# Autodesk Inventor assembly: Cold Plate
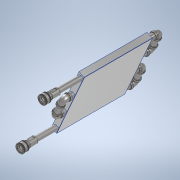
[picture p0: Inventor's stored thumbnail of the model, 180x180]
Saved by Autodesk Inventor 2022 (Build 260153000, 153)
## iProperties
Created: 2022-01-20
Part Number: Cold Plate
Document SubType Name: Assembly
Designer: Caleb
Author: Caleb
## Documents named in this file (8)
- C:\Users\Caleb\Desktop\nebraska-silicon-lab\Hardware\TFPX\Cold Plate\Cold Plate.iam
- C:\Users\Caleb\Desktop\nebraska-silicon-lab\Hardware\TFPX\Cold Plate\43685K12_Low-Pressure Socket-Connect Unthreaded Pipe Fitting.ipt
- C:\Users\Caleb\Desktop\nebraska-silicon-lab\Hardware\TFPX\Cold Plate\outer pipe section.ipt
- C:\Users\Caleb\Desktop\nebraska-silicon-lab\Hardware\TFPX\Cold Plate\inner pipe section.ipt
- C:\Users\Caleb\Desktop\nebraska-silicon-lab\Hardware\TFPX\Cold Plate\Plate.ipt
- C:\Users\Caleb\Desktop\nebraska-silicon-lab\Hardware\TFPX\Cold Plate\5341K26_Pioneer Quick-Disconnect Hose Coupling for Hydraulic Fluid.ipt
- C:\Users\Caleb\Desktop\nebraska-silicon-lab\Hardware\TFPX\Cold Plate\Cover.ipt
- C:\Users\Caleb\Desktop\nebraska-silicon-lab\Hardware\TFPX\Cold Plate\long inner pipe section threaded.ipt
## Components (17 placed, 7 different names)
1. 43685K12_Low-Pressure Socket-Connect Unthreaded Pipe Fitting:1 — Insert:1, Insert:2, Flush:1
2. outer pipe section:1 — Insert:2, Insert:3
3. outer pipe section:2 — Insert:6, Insert:7
4. inner pipe section:1 — Insert:4, Insert:5, Mate:3
5. inner pipe section:2 — Insert:1, Insert:9
6. 43685K12_Low-Pressure Socket-Connect Unthreaded Pipe Fitting:2 — Insert:3, Flush:1, Insert:4
7. 43685K12_Low-Pressure Socket-Connect Unthreaded Pipe Fitting:3 — Insert:5, Insert:6
8. 43685K12_Low-Pressure Socket-Connect Unthreaded Pipe Fitting:4 — Insert:7, Mate:2, Insert:13
9. 43685K12_Low-Pressure Socket-Connect Unthreaded Pipe Fitting:5 — Insert:9, Insert:10
10. 43685K12_Low-Pressure Socket-Connect Unthreaded Pipe Fitting:6 — Insert:11, Insert:12
11. outer pipe section:3 — Insert:10, Insert:11
12. Plate:1 — Mate:2, Mate:3, Mate:4, Flush:2, Flush:3
13. 5341K26_Pioneer Quick-Disconnect Hose Coupling for Hydraulic Fluid:1 — Insert:14
14. 5341K26_Pioneer Quick-Disconnect Hose Coupling for Hydraulic Fluid:2 — Insert:15
15. long inner pipe section threaded:1 — Insert:12, Insert:14
16. long inner pipe section threaded:2 — Insert:13, Insert:15
17. Cover:1 — Mate:4, Flush:2, Flush:3
## Relationships (20: Insert 14, Flush 3, Mate 3)
- Insert:1: 43685K12_Low-Pressure Socket-Connect Unthreaded Pipe Fitting:1 ↔ inner pipe section:2
- Insert:2: 43685K12_Low-Pressure Socket-Connect Unthreaded Pipe Fitting:1 ↔ outer pipe section:1
- Insert:3: outer pipe section:1 ↔ 43685K12_Low-Pressure Socket-Connect Unthreaded Pipe Fitting:2
- Flush:1: 43685K12_Low-Pressure Socket-Connect Unthreaded Pipe Fitting:1 ↔ 43685K12_Low-Pressure Socket-Connect Unthreaded Pipe Fitting:2
- Insert:4: inner pipe section:1 ↔ 43685K12_Low-Pressure Socket-Connect Unthreaded Pipe Fitting:2
- Insert:5: inner pipe section:1 ↔ 43685K12_Low-Pressure Socket-Connect Unthreaded Pipe Fitting:3
- Insert:6: outer pipe section:2 ↔ 43685K12_Low-Pressure Socket-Connect Unthreaded Pipe Fitting:3
- Insert:7: outer pipe section:2 ↔ 43685K12_Low-Pressure Socket-Connect Unthreaded Pipe Fitting:4
- Insert:9: inner pipe section:2 ↔ 43685K12_Low-Pressure Socket-Connect Unthreaded Pipe Fitting:5
- Insert:10: 43685K12_Low-Pressure Socket-Connect Unthreaded Pipe Fitting:5 ↔ outer pipe section:3
- Insert:11: 43685K12_Low-Pressure Socket-Connect Unthreaded Pipe Fitting:6 ↔ outer pipe section:3
- Mate:2 (20.32 mm): 43685K12_Low-Pressure Socket-Connect Unthreaded Pipe Fitting:4 ↔ Plate:1
- Mate:3: inner pipe section:1 ↔ Plate:1
- Insert:12: 43685K12_Low-Pressure Socket-Connect Unthreaded Pipe Fitting:6 ↔ long inner pipe section threaded:1
- Insert:13: 43685K12_Low-Pressure Socket-Connect Unthreaded Pipe Fitting:4 ↔ long inner pipe section threaded:2
- Insert:14: 5341K26_Pioneer Quick-Disconnect Hose Coupling for Hydraulic Fluid:1 ↔ long inner pipe section threaded:1
- Insert:15: 5341K26_Pioneer Quick-Disconnect Hose Coupling for Hydraulic Fluid:2 ↔ long inner pipe section threaded:2
- Mate:4: Plate:1 ↔ Cover:1
- Flush:2: Plate:1 ↔ Cover:1
- Flush:3: Plate:1 ↔ Cover:1
